# Autodesk Inventor assembly: SCARA
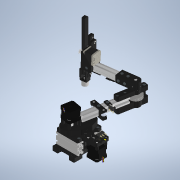
[picture p0: Inventor's stored thumbnail of the model, 180x180]
Saved by Autodesk Inventor 2022 (Build 260153000, 153)
## iProperties
Created: 2022-03-02
Part Number: SCARA
Document SubType Name: Assembly
Designer: JK
Author: JK
## Documents named in this file (4)
- C:\Users\JK\Documents\Inventor\ScaraNema\SCARA-3DP\Parts\SCARA.iam
- C:\Users\JK\Documents\Inventor\ScaraNema\SCARA-3DP\Parts\Shoulder\Shoulder base.iam
- C:\Users\JK\Documents\Inventor\ScaraNema\SCARA-3DP\Parts\Forearm\Forearm assembly.iam
- C:\Users\JK\Documents\Inventor\ScaraNema\SCARA-3DP\Parts\Arm\Arm Assembly.iam
## Components (3 placed, 3 different names)
1. Shoulder base:1 [sub-assembly] — Coincidencia:2, Coincidencia:3
2. Forearm assembly:1 [sub-assembly] — Coincidencia:1, Coincidencia:5
3. Arm Assembly:1 [sub-assembly] — Coincidencia:1, Coincidencia:2, Coincidencia:3, Coincidencia:5
## Relationships (4: Mate 4)
- Coincidencia:1 [Mate]: Forearm assembly:1 ↔ Arm Assembly:1
- Coincidencia:2 [Mate]: Shoulder base:1 ↔ Arm Assembly:1
- Coincidencia:3 [Mate]: Shoulder base:1 ↔ Arm Assembly:1
- Coincidencia:5 [Mate]: Forearm assembly:1 ↔ Arm Assembly:1
